# Autodesk Inventor assembly: ILOHA_Frame
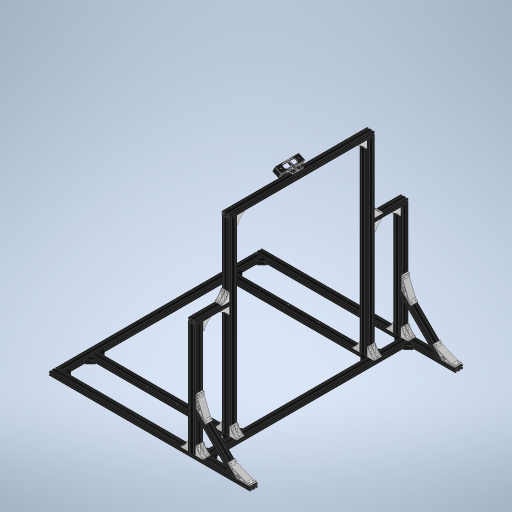
[picture p0: Inventor's stored thumbnail of the model, 512x512]
Saved by Autodesk Inventor 2024.3 (Build 283343010, 343A)
## iProperties
Created: 2026-05-04
Part Number: ILOHA_Frame
Document SubType Name: Assembly
Designer: kshau
Author: kshau
## Documents named in this file (15)
- C:\Users\kshau\Documents\inventor\Create_ViperX\Create_ViperX_ALOHA\ILOHA_Frame.iam
- C:\Users\kshau\Documents\inventor\Create_ViperX\Create_ViperX_ALOHA\NessesaryParts\HFSB5-2040-1053.5\HFSB5-2040-1053.5\HFSB5-2040-1053.5.ipt
- C:\Users\kshau\Documents\inventor\Create_ViperX\Create_ViperX_ALOHA\NessesaryParts\HFSB5-2040-1070\HFSB5-2040-1070\HFSB5-2040-1070.ipt
- C:\Users\kshau\Documents\inventor\Create_ViperX\Create_ViperX_ALOHA\NessesaryParts\HFSB5-4040-600\HFSB5-4040-600\HFSB5-4040-600.ipt
- C:\Users\kshau\Documents\inventor\Create_ViperX\Create_ViperX_ALOHA\NessesaryParts\HFSB5-2040-180\HFSB5-2040-180\HFSB5-2040-180.ipt
- C:\Users\kshau\Documents\inventor\Create_ViperX\Create_ViperX_ALOHA\NessesaryParts\HFSB5-4040-1000\HFSB5-4040-1000\HFSB5-4040-1000.ipt
- C:\Users\kshau\Documents\inventor\Create_ViperX\Create_ViperX_ALOHA\NessesaryParts\HFSB5-2040-305-LBT45-RBT45\HFSB5-2040-305-LBT45-RBT45\HFSB5-2040-305-LBT45-RBT45.ipt
- C:\Users\kshau\Documents\inventor\Create_ViperX\Create_ViperX_ALOHA\NessesaryParts\HBLFSNB5\HBLFSNB5\HBLFSNB5.ipt
- C:\Users\kshau\Documents\inventor\Create_ViperX\Create_ViperX_ALOHA\NessesaryParts\HBLFSDW5\HBLFSDW5\HBLFSDW5.ipt
- C:\Users\kshau\Documents\inventor\Create_ViperX\Create_ViperX_ALOHA\NessesaryParts\HBL135TD5\HBL135TD5\HBL135TD5.ipt
- C:\Users\kshau\Documents\inventor\Create_ViperX\Create_ViperX_ALOHA\overheadcameramount.ipt
- C:\Users\kshau\Documents\inventor\Create_ViperX\Create_ViperX_ALOHA\NessesaryParts\Intel Realsense D455\Intel Realsense D455\Intel Realsense D455.iam
- C:\Users\kshau\Documents\inventor\Create_ViperX\Create_ViperX_ALOHA\NessesaryParts\HFSB5-2040-740-AH290-BH450\HFSB5-2040-740-AH290-BH450\HFSB5-2040-740-AH290-BH450.ipt
- C:\Users\kshau\Documents\inventor\Create_ViperX\Create_ViperX_ALOHA\NessesaryParts\HFSB5-2040-773.5-AH366-BH407.5\HFSB5-2040-773.5-AH366-BH407.5\HFSB5-2040-773.5-AH366-BH407.5.ipt
- C:\Users\kshau\Documents\inventor\Create_ViperX\Create_ViperX_ALOHA\spacer_for_frame.ipt
## Components (57 placed, 14 different names)
1. HFSB5-2040-1053.5:1 — フラッシュ:1, フラッシュ:2, メイト:7, メイト:9, メイト:12, メイト:22, メイト:24, メイト:27, メイト:31, メイト:38, メイト:41, メイト:43, メイト:44, メイト:52, メイト:56, メイト:88, メイト:94
2. HFSB5-2040-1053.5:2 — フラッシュ:1, フラッシュ:2, フラッシュ:3, メイト:1, フラッシュ:4, フラッシュ:5, メイト:2, フラッシュ:6, メイト:19, メイト:21, メイト:29, メイト:32, メイト:35, メイト:36, フラッシュ:62, フラッシュ:64
3. HFSB5-2040-1070:1 — フラッシュ:3, メイト:1, フラッシュ:4, フラッシュ:12, メイト:15, フラッシュ:24, メイト:18, メイト:23, メイト:45, メイト:47, メイト:49, メイト:78
4. HFSB5-2040-1070:2 — フラッシュ:5, メイト:2, フラッシュ:6, メイト:6, フラッシュ:9, メイト:16, メイト:34, メイト:40, メイト:42, フラッシュ:39, メイト:55, メイト:60, メイト:83, フラッシュ:59
5. HFSB5-4040-600:1 — メイト:6, フラッシュ:9, フラッシュ:10, フラッシュ:11, メイト:7, フラッシュ:13, フラッシュ:14, メイト:8, メイト:17, フラッシュ:25, メイト:54, メイト:61, フラッシュ:40, フラッシュ:41, メイト:76, フラッシュ:48, メイト:84
6. HFSB5-4040-600:2 — フラッシュ:10, フラッシュ:11, フラッシュ:12, フラッシュ:17, フラッシュ:18, メイト:14, メイト:46, メイト:48, フラッシュ:46, フラッシュ:47, メイト:65, フラッシュ:55, メイト:80
7. HFSB5-2040-180:1 — フラッシュ:13, フラッシュ:14, メイト:8, フラッシュ:15, フラッシュ:16, メイト:11, フラッシュ:20, メイト:72, メイト:75, メイト:77
8. HFSB5-2040-180:2 — フラッシュ:15, フラッシュ:16, フラッシュ:17, メイト:10, メイト:62, メイト:64, メイト:66
9. HFSB5-4040-1000:1 — メイト:9, フラッシュ:18, メイト:10, メイト:50, メイト:53, フラッシュ:44, フラッシュ:45, メイト:63, メイト:67, メイト:69, フラッシュ:52, フラッシュ:53, フラッシュ:54, フラッシュ:61
10. HFSB5-4040-1000:2 — メイト:11, フラッシュ:20, メイト:12, メイト:57, メイト:58, フラッシュ:42, フラッシュ:43, メイト:71, メイト:73, メイト:74, フラッシュ:49, フラッシュ:50, フラッシュ:51, フラッシュ:63, メイト:100, フラッシュ:65, フラッシュ:66
11. HFSB5-2040-305-LBT45-RBT45:1 — メイト:14, メイト:15, フラッシュ:24, メイト:79, メイト:81, フラッシュ:58
12. HFSB5-2040-305-LBT45-RBT45:2 — メイト:16, メイト:17, フラッシュ:25, メイト:82, メイト:85
13. HBLFSNB5:1 — メイト:31, フラッシュ:30, フラッシュ:31, メイト:97
14. HBLFSNB5:2 — メイト:32, フラッシュ:29, フラッシュ:30, メイト:98
15. HBLFSNB5:3 — メイト:34, メイト:35, フラッシュ:28
16. HBLFSNB5:4 — メイト:36, フラッシュ:27, フラッシュ:28, フラッシュ:29, メイト:99
17. HBLFSNB5:5 — メイト:29, フラッシュ:36, メイト:90
18. HBLFSNB5:6 — メイト:18, メイト:19, フラッシュ:34, フラッシュ:35
19. HBLFSNB5:7 — メイト:22, メイト:23, フラッシュ:33, フラッシュ:34, フラッシュ:37
20. HBLFSNB5:8 — メイト:27, フラッシュ:31, フラッシュ:32, メイト:93
21. HBLFSNB5:9 — メイト:38, フラッシュ:26, フラッシュ:27, メイト:96
22. HBLFSNB5:10 — メイト:40, メイト:41, フラッシュ:26
23. HBLFSNB5:11 — メイト:24, フラッシュ:32, フラッシュ:33, メイト:92
24. HBLFSNB5:12 — メイト:21, フラッシュ:35, フラッシュ:36
25. HBLFSNB5:13 — メイト:44, メイト:45, フラッシュ:37, フラッシュ:38
26. HBLFSNB5:14 — メイト:42, メイト:43, フラッシュ:38, フラッシュ:39
27. HBLFSDW5:1 — メイト:52, メイト:53, フラッシュ:45
28. HBLFSDW5:2 — メイト:46, メイト:47, フラッシュ:47
29. HBLFSDW5:3 — メイト:56, メイト:57, フラッシュ:43
30. HBLFSDW5:4 — メイト:54, メイト:55, フラッシュ:41
31. HBLFSDW5:5 — メイト:48, メイト:49, フラッシュ:46
32. HBLFSDW5:6 — メイト:50, フラッシュ:44, メイト:89, メイト:91
33. HBLFSDW5:7 — メイト:60, メイト:61, フラッシュ:40
34. HBLFSDW5:8 — メイト:58, フラッシュ:42, メイト:95
35. HBLFSDW5:9 — メイト:66, メイト:67, フラッシュ:53
36. HBLFSDW5:10 — メイト:62, メイト:63, フラッシュ:54
37. HBLFSDW5:11 — メイト:64, メイト:65, フラッシュ:55
38. HBLFSDW5:12 — メイト:69, フラッシュ:52, メイト:102
39. HBLFSDW5:13 — メイト:72, メイト:73, フラッシュ:50
40. HBLFSDW5:14 — メイト:76, メイト:77, フラッシュ:48
41. HBLFSDW5:15 — メイト:71, フラッシュ:51, フラッシュ:67, メイト:101
42. HBLFSDW5:16 — メイト:74, メイト:75, フラッシュ:49
43. HBL135TD5:1 — メイト:78, メイト:81, フラッシュ:57
44. HBL135TD5:2 — メイト:82, メイト:83, フラッシュ:56, フラッシュ:59
45. HBL135TD5:3 — メイト:84, メイト:85, フラッシュ:56
46. HBL135TD5:4 — メイト:79, メイト:80, フラッシュ:57, フラッシュ:58
47. overheadcameramount:1 — 回転:1, 回転:2, メイト:103, メイト:104, メイト:105, 回転:3, 回転:4
48. Intel Realsense D455:1 [sub-assembly] — 回転:1, 回転:2
49. HFSB5-2040-740-AH290-BH450:1 — メイト:88, メイト:89, フラッシュ:61, メイト:90, メイト:91, メイト:92, メイト:93, フラッシュ:64, メイト:106, フラッシュ:68, フラッシュ:69, メイト:107
50. HFSB5-2040-740-AH290-BH450:2 — メイト:94, フラッシュ:62, フラッシュ:63, メイト:95, メイト:96, メイト:97, メイト:98, メイト:99, メイト:108, メイト:109, フラッシュ:70, フラッシュ:71
51. HFSB5-2040-773.5-AH366-BH407.5:1 — メイト:100, フラッシュ:65, フラッシュ:66, フラッシュ:67, メイト:101, メイト:102, メイト:103, メイト:104, メイト:105
52. spacer_for_frame:1 — メイト:106, フラッシュ:68
53. spacer_for_frame:2 — フラッシュ:69, メイト:107
54. spacer_for_frame:3 — メイト:108, フラッシュ:71
55. spacer_for_frame:4 — メイト:109, フラッシュ:70
56. spacer_for_frame:5 — 回転:3
57. spacer_for_frame:6 — 回転:4
## Relationships (159: Mate 91, Flush 64, RevoluteJoint 4)
- フラッシュ:1 [Flush]: HFSB5-2040-1053.5:1 ↔ HFSB5-2040-1053.5:2
- フラッシュ:2 [Flush]: HFSB5-2040-1053.5:1 ↔ HFSB5-2040-1053.5:2
- フラッシュ:3 [Flush]: HFSB5-2040-1053.5:2 ↔ HFSB5-2040-1070:1
- メイト:1 [Mate]: HFSB5-2040-1053.5:2 ↔ HFSB5-2040-1070:1
- フラッシュ:4 [Flush]: HFSB5-2040-1053.5:2 ↔ HFSB5-2040-1070:1
- フラッシュ:5 [Flush]: HFSB5-2040-1053.5:2 ↔ HFSB5-2040-1070:2
- メイト:2 [Mate]: HFSB5-2040-1053.5:2 ↔ HFSB5-2040-1070:2
- フラッシュ:6 [Flush]: HFSB5-2040-1053.5:2 ↔ HFSB5-2040-1070:2
- メイト:6 [Mate]: HFSB5-2040-1070:2 ↔ HFSB5-4040-600:1
- フラッシュ:9 [Flush]: HFSB5-2040-1070:2 ↔ HFSB5-4040-600:1
- フラッシュ:10 [Flush]: HFSB5-4040-600:1 ↔ HFSB5-4040-600:2
- フラッシュ:11 [Flush]: HFSB5-4040-600:1 ↔ HFSB5-4040-600:2
- フラッシュ:12 [Flush]: HFSB5-2040-1070:1 ↔ HFSB5-4040-600:2
- メイト:7 [Mate]: HFSB5-2040-1053.5:1 ↔ HFSB5-4040-600:1
- フラッシュ:13 [Flush]: HFSB5-4040-600:1 ↔ HFSB5-2040-180:1
- フラッシュ:14 [Flush]: HFSB5-4040-600:1 ↔ HFSB5-2040-180:1
- メイト:8 [Mate]: HFSB5-4040-600:1 ↔ HFSB5-2040-180:1
- フラッシュ:15 [Flush]: HFSB5-2040-180:1 ↔ HFSB5-2040-180:2
- フラッシュ:16 [Flush]: HFSB5-2040-180:1 ↔ HFSB5-2040-180:2
- フラッシュ:17 [Flush]: HFSB5-4040-600:2 ↔ HFSB5-2040-180:2
- メイト:9 [Mate]: HFSB5-2040-1053.5:1 ↔ HFSB5-4040-1000:1
- フラッシュ:18 [Flush]: HFSB5-4040-600:2 ↔ HFSB5-4040-1000:1
- メイト:10 [Mate]: HFSB5-2040-180:2 ↔ HFSB5-4040-1000:1
- メイト:11 [Mate]: HFSB5-2040-180:1 ↔ HFSB5-4040-1000:2
- フラッシュ:20 [Flush]: HFSB5-2040-180:1 ↔ HFSB5-4040-1000:2
- メイト:12 [Mate]: HFSB5-2040-1053.5:1 ↔ HFSB5-4040-1000:2
- メイト:14 [Mate]: HFSB5-4040-600:2 ↔ HFSB5-2040-305-LBT45-RBT45:1
- メイト:15 [Mate]: HFSB5-2040-1070:1 ↔ HFSB5-2040-305-LBT45-RBT45:1
- フラッシュ:24 [Flush]: HFSB5-2040-1070:1 ↔ HFSB5-2040-305-LBT45-RBT45:1
- メイト:16 [Mate]: HFSB5-2040-1070:2 ↔ HFSB5-2040-305-LBT45-RBT45:2
- メイト:17 [Mate]: HFSB5-4040-600:1 ↔ HFSB5-2040-305-LBT45-RBT45:2
- フラッシュ:25 [Flush]: HFSB5-4040-600:1 ↔ HFSB5-2040-305-LBT45-RBT45:2
- メイト:18 [Mate]: HFSB5-2040-1070:1 ↔ HBLFSNB5:6
- メイト:19 [Mate]: HFSB5-2040-1053.5:2 ↔ HBLFSNB5:6
- メイト:21 [Mate]: HFSB5-2040-1053.5:2 ↔ HBLFSNB5:12
- メイト:22 [Mate]: HFSB5-2040-1053.5:1 ↔ HBLFSNB5:7
- メイト:23 [Mate]: HFSB5-2040-1070:1 ↔ HBLFSNB5:7
- メイト:24 [Mate]: HFSB5-2040-1053.5:1 ↔ HBLFSNB5:11
- メイト:27 [Mate]: HFSB5-2040-1053.5:1 ↔ HBLFSNB5:8
- メイト:29 [Mate]: HFSB5-2040-1053.5:2 ↔ HBLFSNB5:5
- メイト:31 [Mate]: HFSB5-2040-1053.5:1 ↔ HBLFSNB5:1
- メイト:32 [Mate]: HFSB5-2040-1053.5:2 ↔ HBLFSNB5:2
- メイト:34 [Mate]: HFSB5-2040-1070:2 ↔ HBLFSNB5:3
- メイト:35 [Mate]: HFSB5-2040-1053.5:2 ↔ HBLFSNB5:3
- メイト:36 [Mate]: HFSB5-2040-1053.5:2 ↔ HBLFSNB5:4
- メイト:38 [Mate]: HFSB5-2040-1053.5:1 ↔ HBLFSNB5:9
- メイト:40 [Mate]: HFSB5-2040-1070:2 ↔ HBLFSNB5:10
- メイト:41 [Mate]: HFSB5-2040-1053.5:1 ↔ HBLFSNB5:10
- フラッシュ:26 [Flush]: HBLFSNB5:9 ↔ HBLFSNB5:10
- フラッシュ:27 [Flush]: HBLFSNB5:4 ↔ HBLFSNB5:9
- フラッシュ:28 [Flush]: HBLFSNB5:3 ↔ HBLFSNB5:4
- フラッシュ:29 [Flush]: HBLFSNB5:2 ↔ HBLFSNB5:4
- フラッシュ:30 [Flush]: HBLFSNB5:1 ↔ HBLFSNB5:2
- フラッシュ:31 [Flush]: HBLFSNB5:1 ↔ HBLFSNB5:8
- フラッシュ:32 [Flush]: HBLFSNB5:8 ↔ HBLFSNB5:11
- フラッシュ:33 [Flush]: HBLFSNB5:7 ↔ HBLFSNB5:11
- フラッシュ:34 [Flush]: HBLFSNB5:6 ↔ HBLFSNB5:7
- フラッシュ:35 [Flush]: HBLFSNB5:6 ↔ HBLFSNB5:12
- フラッシュ:36 [Flush]: HBLFSNB5:5 ↔ HBLFSNB5:12
- メイト:42 [Mate]: HFSB5-2040-1070:2 ↔ HBLFSNB5:14
- メイト:43 [Mate]: HFSB5-2040-1053.5:1 ↔ HBLFSNB5:14
- メイト:44 [Mate]: HFSB5-2040-1053.5:1 ↔ HBLFSNB5:13
- メイト:45 [Mate]: HFSB5-2040-1070:1 ↔ HBLFSNB5:13
- フラッシュ:37 [Flush]: HBLFSNB5:7 ↔ HBLFSNB5:13
- フラッシュ:38 [Flush]: HBLFSNB5:13 ↔ HBLFSNB5:14
- フラッシュ:39 [Flush]: HFSB5-2040-1070:2 ↔ HBLFSNB5:14
- メイト:46 [Mate]: HFSB5-4040-600:2 ↔ HBLFSDW5:2
- メイト:47 [Mate]: HFSB5-2040-1070:1 ↔ HBLFSDW5:2
- メイト:48 [Mate]: HFSB5-4040-600:2 ↔ HBLFSDW5:5
- メイト:49 [Mate]: HFSB5-2040-1070:1 ↔ HBLFSDW5:5
- メイト:50 [Mate]: HFSB5-4040-1000:1 ↔ HBLFSDW5:6
- メイト:52 [Mate]: HFSB5-2040-1053.5:1 ↔ HBLFSDW5:1
- メイト:53 [Mate]: HFSB5-4040-1000:1 ↔ HBLFSDW5:1
- メイト:54 [Mate]: HFSB5-4040-600:1 ↔ HBLFSDW5:4
- メイト:55 [Mate]: HFSB5-2040-1070:2 ↔ HBLFSDW5:4
- メイト:56 [Mate]: HFSB5-2040-1053.5:1 ↔ HBLFSDW5:3
- メイト:57 [Mate]: HFSB5-4040-1000:2 ↔ HBLFSDW5:3
- メイト:58 [Mate]: HFSB5-4040-1000:2 ↔ HBLFSDW5:8
- メイト:60 [Mate]: HFSB5-2040-1070:2 ↔ HBLFSDW5:7
- メイト:61 [Mate]: HFSB5-4040-600:1 ↔ HBLFSDW5:7
- フラッシュ:40 [Flush]: HFSB5-4040-600:1 ↔ HBLFSDW5:7
- フラッシュ:41 [Flush]: HFSB5-4040-600:1 ↔ HBLFSDW5:4
- フラッシュ:42 [Flush]: HFSB5-4040-1000:2 ↔ HBLFSDW5:8
- フラッシュ:43 [Flush]: HFSB5-4040-1000:2 ↔ HBLFSDW5:3
- フラッシュ:44 [Flush]: HFSB5-4040-1000:1 ↔ HBLFSDW5:6
- フラッシュ:45 [Flush]: HFSB5-4040-1000:1 ↔ HBLFSDW5:1
- フラッシュ:46 [Flush]: HFSB5-4040-600:2 ↔ HBLFSDW5:5
- フラッシュ:47 [Flush]: HFSB5-4040-600:2 ↔ HBLFSDW5:2
- メイト:62 [Mate]: HFSB5-2040-180:2 ↔ HBLFSDW5:10
- メイト:63 [Mate]: HFSB5-4040-1000:1 ↔ HBLFSDW5:10
- メイト:64 [Mate]: HFSB5-2040-180:2 ↔ HBLFSDW5:11
- メイト:65 [Mate]: HFSB5-4040-600:2 ↔ HBLFSDW5:11
- メイト:66 [Mate]: HFSB5-2040-180:2 ↔ HBLFSDW5:9
- メイト:67 [Mate]: HFSB5-4040-1000:1 ↔ HBLFSDW5:9
- メイト:69 [Mate]: HFSB5-4040-1000:1 ↔ HBLFSDW5:12
- メイト:71 [Mate]: HFSB5-4040-1000:2 ↔ HBLFSDW5:15
- メイト:72 [Mate]: HFSB5-2040-180:1 ↔ HBLFSDW5:13
- メイト:73 [Mate]: HFSB5-4040-1000:2 ↔ HBLFSDW5:13
- メイト:74 [Mate]: HFSB5-4040-1000:2 ↔ HBLFSDW5:16
- メイト:75 [Mate]: HFSB5-2040-180:1 ↔ HBLFSDW5:16
- メイト:76 [Mate]: HFSB5-4040-600:1 ↔ HBLFSDW5:14
- メイト:77 [Mate]: HFSB5-2040-180:1 ↔ HBLFSDW5:14
- フラッシュ:48 [Flush]: HFSB5-4040-600:1 ↔ HBLFSDW5:14
- フラッシュ:49 [Flush]: HFSB5-4040-1000:2 ↔ HBLFSDW5:16
- フラッシュ:50 [Flush]: HFSB5-4040-1000:2 ↔ HBLFSDW5:13
- フラッシュ:51 [Flush]: HFSB5-4040-1000:2 ↔ HBLFSDW5:15
- フラッシュ:52 [Flush]: HFSB5-4040-1000:1 ↔ HBLFSDW5:12
- フラッシュ:53 [Flush]: HFSB5-4040-1000:1 ↔ HBLFSDW5:9
- フラッシュ:54 [Flush]: HFSB5-4040-1000:1 ↔ HBLFSDW5:10
- フラッシュ:55 [Flush]: HFSB5-4040-600:2 ↔ HBLFSDW5:11
- メイト:78 [Mate]: HFSB5-2040-1070:1 ↔ HBL135TD5:1
- メイト:79 [Mate]: HFSB5-2040-305-LBT45-RBT45:1 ↔ HBL135TD5:4
- メイト:80 [Mate]: HFSB5-4040-600:2 ↔ HBL135TD5:4
- メイト:81 [Mate]: HFSB5-2040-305-LBT45-RBT45:1 ↔ HBL135TD5:1
- メイト:82 [Mate]: HFSB5-2040-305-LBT45-RBT45:2 ↔ HBL135TD5:2
- メイト:83 [Mate]: HFSB5-2040-1070:2 ↔ HBL135TD5:2
- メイト:84 [Mate]: HFSB5-4040-600:1 ↔ HBL135TD5:3
- メイト:85 [Mate]: HFSB5-2040-305-LBT45-RBT45:2 ↔ HBL135TD5:3
- フラッシュ:56 [Flush]: HBL135TD5:2 ↔ HBL135TD5:3
- フラッシュ:57 [Flush]: HBL135TD5:1 ↔ HBL135TD5:4
- フラッシュ:58 [Flush] (3 mm): HFSB5-2040-305-LBT45-RBT45:1 ↔ HBL135TD5:4
- フラッシュ:59 [Flush] (3 mm): HFSB5-2040-1070:2 ↔ HBL135TD5:2
- 回転:1 [RevoluteJoint]: overheadcameramount:1 ↔ Intel Realsense D455:1
- 回転:2 [RevoluteJoint]: overheadcameramount:1 ↔ Intel Realsense D455:1
- メイト:88 [Mate]: HFSB5-2040-1053.5:1 ↔ HFSB5-2040-740-AH290-BH450:1
- メイト:89 [Mate]: HBLFSDW5:6 ↔ HFSB5-2040-740-AH290-BH450:1
- フラッシュ:61 [Flush]: HFSB5-4040-1000:1 ↔ HFSB5-2040-740-AH290-BH450:1
- メイト:90 [Mate]: HBLFSNB5:5 ↔ HFSB5-2040-740-AH290-BH450:1
- メイト:91 [Mate]: HBLFSDW5:6 ↔ HFSB5-2040-740-AH290-BH450:1
- メイト:92 [Mate]: HBLFSNB5:11 ↔ HFSB5-2040-740-AH290-BH450:1
- メイト:93 [Mate]: HBLFSNB5:8 ↔ HFSB5-2040-740-AH290-BH450:1
- メイト:94 [Mate]: HFSB5-2040-1053.5:1 ↔ HFSB5-2040-740-AH290-BH450:2
- フラッシュ:62 [Flush]: HFSB5-2040-1053.5:2 ↔ HFSB5-2040-740-AH290-BH450:2
- フラッシュ:63 [Flush]: HFSB5-4040-1000:2 ↔ HFSB5-2040-740-AH290-BH450:2
- メイト:95 [Mate]: HBLFSDW5:8 ↔ HFSB5-2040-740-AH290-BH450:2
- メイト:96 [Mate]: HBLFSNB5:9 ↔ HFSB5-2040-740-AH290-BH450:2
- メイト:97 [Mate]: HBLFSNB5:1 ↔ HFSB5-2040-740-AH290-BH450:2
- メイト:98 [Mate]: HBLFSNB5:2 ↔ HFSB5-2040-740-AH290-BH450:2
- メイト:99 [Mate]: HBLFSNB5:4 ↔ HFSB5-2040-740-AH290-BH450:2
- フラッシュ:64 [Flush]: HFSB5-2040-1053.5:2 ↔ HFSB5-2040-740-AH290-BH450:1
- メイト:100 [Mate]: HFSB5-4040-1000:2 ↔ HFSB5-2040-773.5-AH366-BH407.5:1
- フラッシュ:65 [Flush]: HFSB5-4040-1000:2 ↔ HFSB5-2040-773.5-AH366-BH407.5:1
- フラッシュ:66 [Flush]: HFSB5-4040-1000:2 ↔ HFSB5-2040-773.5-AH366-BH407.5:1
- フラッシュ:67 [Flush]: HBLFSDW5:15 ↔ HFSB5-2040-773.5-AH366-BH407.5:1
- メイト:101 [Mate]: HBLFSDW5:15 ↔ HFSB5-2040-773.5-AH366-BH407.5:1
- メイト:102 [Mate]: HBLFSDW5:12 ↔ HFSB5-2040-773.5-AH366-BH407.5:1
- メイト:103 [Mate]: overheadcameramount:1 ↔ HFSB5-2040-773.5-AH366-BH407.5:1
- メイト:104 [Mate]: overheadcameramount:1 ↔ HFSB5-2040-773.5-AH366-BH407.5:1
- メイト:105 [Mate]: overheadcameramount:1 ↔ HFSB5-2040-773.5-AH366-BH407.5:1
- メイト:106 [Mate]: HFSB5-2040-740-AH290-BH450:1 ↔ spacer_for_frame:1
- フラッシュ:68 [Flush]: HFSB5-2040-740-AH290-BH450:1 ↔ spacer_for_frame:1
- フラッシュ:69 [Flush]: HFSB5-2040-740-AH290-BH450:1 ↔ spacer_for_frame:2
- メイト:107 [Mate]: HFSB5-2040-740-AH290-BH450:1 ↔ spacer_for_frame:2
- メイト:108 [Mate]: HFSB5-2040-740-AH290-BH450:2 ↔ spacer_for_frame:3
- メイト:109 [Mate]: HFSB5-2040-740-AH290-BH450:2 ↔ spacer_for_frame:4
- フラッシュ:70 [Flush]: HFSB5-2040-740-AH290-BH450:2 ↔ spacer_for_frame:4
- フラッシュ:71 [Flush]: HFSB5-2040-740-AH290-BH450:2 ↔ spacer_for_frame:3
- 回転:3 [RevoluteJoint]: overheadcameramount:1 ↔ spacer_for_frame:5
- 回転:4 [RevoluteJoint]: overheadcameramount:1 ↔ spacer_for_frame:6
